# Autodesk Inventor assembly: Granny Gear Layout
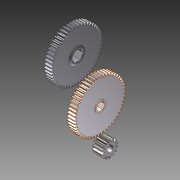
[picture p0: Inventor's stored thumbnail of the model, 180x180]
Saved by Autodesk Inventor 2015 (Build 190159000, 159)
## iProperties
Created: 2016-02-24
Part Number: Granny Gear Layout
Document SubType Name: Assembly
Designer: sethbattis
Author: sethbattis
## Documents named in this file (5)
- \\area51\team3566\cad\FRC 2016\Tough Box Gears\Granny Gear Layout.iam
- \\area51\team3566\cad\FRC 2016\Tough Box Gears\14T 20dp 375hex_Inch - Spur gear 20DP 14T 14.5PA .568FW ---S14N3.0H2.0L0.25N.ipt
- \\area51\team3566\cad\FRC 2016\Tough Box Gears\14T CIM Gear.ipt
- \\area51\team3566\cad\FRC 2016\Tough Box Gears\50T 20dp 375hex_Inch - Spur gear 20DP 50T 14.5PA .372FW ---S50N3.0H2.0L0.25N.ipt
- \\area51\team3566\cad\FRC 2016\Tough Box Gears\50T 20dp 500hex.ipt
## Components (4 placed, 4 different names)
1. 14T 20dp 375hex_Inch - Spur gear 20DP 14T 14.5PA .568FW ---S14N3.0H2.0L0.25N:1 — Flush:1, Mate:1, Flush:2, Flush:3
2. 14T CIM Gear:1
3. 50T 20dp 375hex_Inch - Spur gear 20DP 50T 14.5PA .372FW ---S50N3.0H2.0L0.25N:1 — Flush:1, Mate:1, Flush:2, Flush:3
4. 50T 20dp 500hex:1
## Relationships (4: Flush 3, Mate 1)
- Flush:1: 14T 20dp 375hex_Inch - Spur gear 20DP 14T 14.5PA .568FW ---S14N3.0H2.0L0.25N:1 ↔ 50T 20dp 375hex_Inch - Spur gear 20DP 50T 14.5PA .372FW ---S50N3.0H2.0L0.25N:1
- Mate:1: 14T 20dp 375hex_Inch - Spur gear 20DP 14T 14.5PA .568FW ---S14N3.0H2.0L0.25N:1 ↔ 50T 20dp 375hex_Inch - Spur gear 20DP 50T 14.5PA .372FW ---S50N3.0H2.0L0.25N:1
- Flush:2: 14T 20dp 375hex_Inch - Spur gear 20DP 14T 14.5PA .568FW ---S14N3.0H2.0L0.25N:1 ↔ 50T 20dp 375hex_Inch - Spur gear 20DP 50T 14.5PA .372FW ---S50N3.0H2.0L0.25N:1
- Flush:3: 14T 20dp 375hex_Inch - Spur gear 20DP 14T 14.5PA .568FW ---S14N3.0H2.0L0.25N:1 ↔ 50T 20dp 375hex_Inch - Spur gear 20DP 50T 14.5PA .372FW ---S50N3.0H2.0L0.25N:1
